# Autodesk Inventor assembly: Chuck Assembly
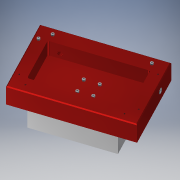
[picture p0: Inventor's stored thumbnail of the model, 180x180]
Saved by Autodesk Inventor 2019.4 (Build 234330000, 330)
## iProperties
Created: 2021-01-20
Part Number: Chuck Assembly
Document SubType Name: Assembly
Designer: caleb
Author: caleb
## Documents named in this file (7)
- C:\Users\cfang\Desktop\nebraska-silicon-lab\CAD\Wirebonder\Chuck Assembly.iam
- C:\Users\cfang\Desktop\nebraska-silicon-lab\CAD\Wirebonder\Chuck.ipt
- C:\Users\cfang\Desktop\nebraska-silicon-lab\CAD\Wirebonder\Chuck Spacer.ipt
- C:\Users\cfang\Desktop\nebraska-silicon-lab\CAD\Wirebonder\90128A211_ZNC-PLTD ALLOY STL SCKT HEAD CAP SCREW.ipt
- C:\Users\cfang\Desktop\nebraska-silicon-lab\CAD\Wirebonder\4464K562_TYPE 304 STAINLESS STL THREADED PIPE FITTING.ipt
- C:\Users\cfang\Desktop\nebraska-silicon-lab\CAD\Wirebonder\44555K151_BRASS BARBED TUBE FITTING FOR VACUUM.ipt
- C:\Users\cfang\Desktop\nebraska-silicon-lab\CAD\Wirebonder\90128A216_ZNC-PLTD ALLOY STL SCKT HEAD CAP SCREW.ipt
## Components (11 placed, 6 different names)
1. Chuck:1 — Mate:1, Angle:1, Insert:1, Insert:2, Insert:3, Insert:4, Insert:5, Insert:6, Insert:7, Insert:8, Insert:9, Insert:10
2. Chuck Spacer:1 — Mate:1, Angle:1, Insert:1
3. 90128A211_ZNC-PLTD ALLOY STL SCKT HEAD CAP SCREW:1 — Insert:4
4. 90128A211_ZNC-PLTD ALLOY STL SCKT HEAD CAP SCREW:2 — Insert:3
5. 90128A211_ZNC-PLTD ALLOY STL SCKT HEAD CAP SCREW:3 — Insert:2
6. 4464K562_TYPE 304 STAINLESS STL THREADED PIPE FITTING:1 — Insert:5
7. 44555K151_BRASS BARBED TUBE FITTING FOR VACUUM:1 — Insert:6
8. 90128A216_ZNC-PLTD ALLOY STL SCKT HEAD CAP SCREW:1 — Insert:10
9. 90128A216_ZNC-PLTD ALLOY STL SCKT HEAD CAP SCREW:2 — Insert:8
10. 90128A216_ZNC-PLTD ALLOY STL SCKT HEAD CAP SCREW:3 — Insert:7
11. 90128A216_ZNC-PLTD ALLOY STL SCKT HEAD CAP SCREW:4 — Insert:9
## Relationships (12: Insert 10, Mate 1, Angle 1)
- Mate:1: Chuck:1 ↔ Chuck Spacer:1
- Angle:1 (0 deg): Chuck:1 ↔ Chuck Spacer:1
- Insert:1: Chuck:1 ↔ Chuck Spacer:1
- Insert:2: Chuck:1 ↔ 90128A211_ZNC-PLTD ALLOY STL SCKT HEAD CAP SCREW:3
- Insert:3: Chuck:1 ↔ 90128A211_ZNC-PLTD ALLOY STL SCKT HEAD CAP SCREW:2
- Insert:4: Chuck:1 ↔ 90128A211_ZNC-PLTD ALLOY STL SCKT HEAD CAP SCREW:1
- Insert:5: Chuck:1 ↔ 4464K562_TYPE 304 STAINLESS STL THREADED PIPE FITTING:1
- Insert:6: Chuck:1 ↔ 44555K151_BRASS BARBED TUBE FITTING FOR VACUUM:1
- Insert:7: Chuck:1 ↔ 90128A216_ZNC-PLTD ALLOY STL SCKT HEAD CAP SCREW:3
- Insert:8: Chuck:1 ↔ 90128A216_ZNC-PLTD ALLOY STL SCKT HEAD CAP SCREW:2
- Insert:9: Chuck:1 ↔ 90128A216_ZNC-PLTD ALLOY STL SCKT HEAD CAP SCREW:4
- Insert:10: Chuck:1 ↔ 90128A216_ZNC-PLTD ALLOY STL SCKT HEAD CAP SCREW:1
